# Autodesk Inventor assembly: X Axis Assembly
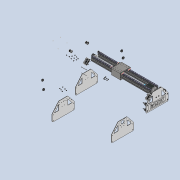
[picture p0: Inventor's stored thumbnail of the model, 180x180]
Saved by Autodesk Inventor 2022 (Build 260153000, 153)
## iProperties
Created: 2021-10-10
Part Number: X Axis Assembly
Document SubType Name: Assembly
Designer: Coy
Author: Coy
## Documents named in this file (23)
- H:\3D Files\Project 3D Models\Breakfast Maker 2000\Assemblys\X Axis Assembly.iam
- H:\3D Files\Project 3D Models\Breakfast Maker 2000\Aluminum Extrusion\2040\2040x700 silver profile.ipt
- H:\3D Files\Project 3D Models\Breakfast Maker 2000\Linear Actuators\MGN12C Linear Rail.iam
- H:\3D Files\Downloaded 3D Files\GrabCad Downloads\hiwin-mgn-series-full-2.snapshot.14\PRODUCT_NAME_10.ipt
- H:\3D Files\Project 3D Models\Breakfast Maker 2000\X Axis V Wheel and Motor Frame Machined.ipt
- H:\3D Files\Project 3D Models\Breakfast Maker 2000\Motors\Nema 23 Dual Shaft 87mm Stepper Motor.ipt
- H:\3D Files\Project 3D Models\Breakfast Maker 2000\X Axis V Wheel Frame Machined.ipt
- H:\3D Files\Project 3D Models\Breakfast Maker 2000\Bearings\0.5in Flanged Pillowblock Frame.ipt
- H:\3D Files\Project 3D Models\Breakfast Maker 2000\Bearings\0.25in ID 0.5in OD 0.1875in Deep Roller Bearing.ipt
- H:\3D Files\Project 3D Models\Breakfast Maker 2000\Shafts and Rods\M6.35 x 356mm Aluminum Rod.ipt
- H:\3D Files\Project 3D Models\Breakfast Maker 2000\Shafts and Rods\M6.35 x 275mm Aluminum Rod.ipt
- H:\3D Files\Project 3D Models\Breakfast Maker 2000\Couplers\M6.35 Rigid Coupler.ipt
- H:\3D Files\Project 3D Models\Breakfast Maker 2000\Pullys\M6.35 24Tooth 15mm Deep 3M Timing Pulley.ipt
- H:\3D Files\Project 3D Models\Breakfast Maker 2000\3in x 5in Steel Rectangular Tubing 4in long.ipt
- H:\3D Files\Project 3D Models\Breakfast Maker 2000\Pullys\8mm ID 15mm Deep Idler Pully.ipt
- H:\3D Files\Project 3D Models\Breakfast Maker 2000\Bearings\5mm ID 8mm OD 2.5mm Deep Roller Bearing (2021_08_15 23_37_01 UTC).ipt
- H:\3D Files\Project 3D Models\Breakfast Maker 2000\X Axis V Wheel Outside Frame Machined.ipt
- H:\3D Files\Project 3D Models\Breakfast Maker 2000\Shafts and Rods\M5 55mm Threaded Rod.ipt
- H:\3D Files\Project 3D Models\Breakfast Maker 2000\X Axis Belt and V Wheel Plate Spacer.ipt
- H:\3D Files\Project 3D Models\Breakfast Maker 2000\Nuts and Bolts\M5 Nut Silver.ipt
- H:\3D Files\Project 3D Models\Breakfast Maker 2000\Idler Pully Spacer.ipt
- H:\3D Files\Project 3D Models\Breakfast Maker 2000\V Wheel Spacer.ipt
- H:\3D Files\Project 3D Models\Breakfast Maker 2000\M5 V Wheel.ipt
## Components (154 placed, 22 different names)
1. 2040x700 silver profile:1 — Flush:1, Flush:2, Mate:2, Mate:4, Flush:6
2. 2040x700 silver profile:2 — Mate:1, Flush:1, Flush:2, Mate:2, Mate:3, Flush:3, Flush:4, Mate:43
3. MGN12C Linear Rail:1 [sub-assembly] — Mate:7, Flush:11, Flush:12, Mate:9, Flush:15, Flush:16, Mate:42
4. MGN12C Linear Rail:2 [sub-assembly] — Mate:8, Flush:13, Flush:14, Mate:10, Flush:17, Flush:18
5. MGN12C Linear Rail:3 [sub-assembly] — Mate:10, Flush:17, Flush:18, Mate:12, Flush:21, Flush:22
6. MGN12C Linear Rail:4 [sub-assembly] — Mate:9, Flush:15, Flush:16, Mate:11, Flush:19, Flush:20
7. PRODUCT_NAME_10:1 — Mate:6, Flush:9, Flush:10, Mate:8, Flush:13, Flush:14
8. PRODUCT_NAME_10:2 — Mate:4, Flush:5, Flush:6, Mate:6, Flush:9, Flush:10
9. PRODUCT_NAME_10:3 — Mate:11, Flush:19, Flush:20, Mate:13, Flush:23, Flush:24
10. PRODUCT_NAME_10:4 — Mate:12, Flush:21, Flush:22, Mate:14, Flush:25, Flush:26
11. PRODUCT_NAME_10:5 — Mate:13, Flush:23, Flush:24, Mate:15, Flush:27, Flush:28
12. PRODUCT_NAME_10:6 — Mate:14, Flush:25, Flush:26, Mate:16, Flush:29, Flush:30
13. PRODUCT_NAME_10:7 — Mate:16, Flush:29, Flush:30
14. PRODUCT_NAME_10:8 — Mate:15, Flush:27, Flush:28
15. PRODUCT_NAME_10:9 — Mate:3, Flush:3, Flush:4, Flush:5, Flush:7, Flush:8, Mate:5
16. PRODUCT_NAME_10:10 — Flush:7, Flush:8, Mate:5, Mate:7, Flush:11, Flush:12
17. Nema 23 Dual Shaft 87mm Stepper Motor:1 — Mate:30, Mate:31, Mate:37, Mate:38, Mate:39, Mate:181
18. 0.5in Flanged Pillowblock Frame:1 — Mate:29, Flush:31
19. 0.25in ID 0.5in OD 0.1875in Deep Roller Bearing:1 — Mate:29, Flush:31
20. M6.35 x 356mm Aluminum Rod:1 — Mate:30, Mate:31, Mate:32, Mate:33, Mate:36
21. M6.35 x 275mm Aluminum Rod:1 — Mate:32, Mate:33, Mate:34, Mate:35, Mate:40
22. M6.35 Rigid Coupler:1 — Mate:34, Mate:35
23. M6.35 Rigid Coupler:2 — Mate:36, Mate:37
24. M6.35 24Tooth 15mm Deep 3M Timing Pulley:1 — Mate:38, Mate:39
25. M6.35 24Tooth 15mm Deep 3M Timing Pulley:2 — Mate:40
26. 3in x 5in Steel Rectangular Tubing 4in long:1 — Mate:42, Mate:43
27. 8mm ID 15mm Deep Idler Pully:1 — Mate:45, Mate:46, Flush:35, Flush:36
28. 8mm ID 15mm Deep Idler Pully:2 — Mate:44, Flush:32, Mate:47, Flush:39
29. 8mm ID 15mm Deep Idler Pully:3 — Mate:48, Mate:51, Flush:33, Flush:37
30. 8mm ID 15mm Deep Idler Pully:4 — Mate:49, Mate:50, Flush:34, Flush:38
31. 5mm ID 8mm OD 2.5mm Deep Roller Bearing (2021_08_15 23_37_01 UTC):1 — Mate:44, Flush:32, Mate:102, Mate:112
32. 5mm ID 8mm OD 2.5mm Deep Roller Bearing (2021_08_15 23_37_01 UTC):2 — Mate:47, Flush:39, Mate:108
33. 5mm ID 8mm OD 2.5mm Deep Roller Bearing (2021_08_15 23_37_01 UTC):3 — Mate:46, Flush:36, Mate:107
34. 5mm ID 8mm OD 2.5mm Deep Roller Bearing (2021_08_15 23_37_01 UTC):4 — Mate:45, Flush:35, Mate:101, Mate:111
35. 5mm ID 8mm OD 2.5mm Deep Roller Bearing (2021_08_15 23_37_01 UTC):5 — Mate:51, Flush:33
36. 5mm ID 8mm OD 2.5mm Deep Roller Bearing (2021_08_15 23_37_01 UTC):6 — Mate:48, Flush:37
37. 5mm ID 8mm OD 2.5mm Deep Roller Bearing (2021_08_15 23_37_01 UTC):7 — Mate:49, Flush:38
38. 5mm ID 8mm OD 2.5mm Deep Roller Bearing (2021_08_15 23_37_01 UTC):8 — Mate:50, Flush:34
39. X Axis V Wheel Outside Frame Machined:1
40. X Axis V Wheel Outside Frame Machined:2 — Mate:165, Mate:166, Mate:167, Mate:178
41. M5 55mm Threaded Rod:1 — Mate:90, Mate:98, Mate:120, Mate:128, Mate:136, Mate:143, Mate:151, Mate:159, Mate:171
42. M5 55mm Threaded Rod:2 — Mate:84, Mate:95, Mate:118, Mate:125, Mate:134, Mate:141, Mate:150, Mate:158, Mate:168
43. M5 55mm Threaded Rod:3 — Mate:91, Mate:99, Mate:119, Mate:127, Mate:135, Mate:144, Mate:152, Mate:160, Mate:165, Mate:169
44. M5 55mm Threaded Rod:4 — Mate:85, Mate:94, Mate:117, Mate:126, Mate:133, Mate:142, Mate:149, Mate:157, Mate:166, Mate:170
45. M5 55mm Threaded Rod:5 — Mate:96, Mate:102, Mate:103, Mate:110, Mate:114, Mate:174, Mate:179
46. M5 55mm Threaded Rod:6 — Mate:97, Mate:101, Mate:104, Mate:109, Mate:113, Mate:175, Mate:180
47. M5 55mm Threaded Rod:7
48. M5 55mm Threaded Rod:8
49. M5 55mm Threaded Rod:9
50. M5 55mm Threaded Rod:10
51. M5 55mm Threaded Rod:11
52. M5 55mm Threaded Rod:12
53. X Axis Belt and V Wheel Plate Spacer:1 — Mate:72, Mate:73, Mate:167
54. X Axis Belt and V Wheel Plate Spacer:2 — Mate:74, Mate:75
55. X Axis Belt and V Wheel Plate Spacer:3 — Mate:76, Mate:77
56. X Axis Belt and V Wheel Plate Spacer:4 — Mate:78, Mate:79
57. M5 55mm Threaded Rod:13 — Mate:72, Mate:87, Mate:172
58. M5 55mm Threaded Rod:14 — Mate:73, Mate:86, Mate:173
59. M5 55mm Threaded Rod:15 — Mate:76
60. M5 55mm Threaded Rod:16 — Mate:79
61. M5 55mm Threaded Rod:17 — Mate:75, Mate:89, Mate:176
62. M5 55mm Threaded Rod:18 — Mate:74, Mate:88, Mate:177
63. M5 55mm Threaded Rod:19 — Mate:77
64. M5 55mm Threaded Rod:20 — Mate:78
65. M5 Nut Silver:1 — Mate:86, Flush:63
66. M5 Nut Silver:2 — Mate:95, Flush:66, Mate:122
67. M5 Nut Silver:3 — Mate:87, Flush:63, Flush:64, Flush:65
68. M5 Nut Silver:4 — Mate:89, Flush:60
69. M5 Nut Silver:5 — Mate:88, Flush:60, Flush:61, Flush:62
70. M5 Nut Silver:6 — Mate:90, Flush:61
71. M5 Nut Silver:7 — Mate:85, Flush:64
72. M5 Nut Silver:8 — Mate:91, Flush:62
73. M5 Nut Silver:9 — Mate:94, Flush:66, Flush:67, Flush:68, Flush:69, Flush:70, Mate:121
74. M5 Nut Silver:10 — Mate:84, Flush:65, Flush:80, Flush:81
75. M5 Nut Silver:11
76. M5 Nut Silver:12
77. M5 Nut Silver:13 — Mate:181
78. M5 Nut Silver:14
79. M5 Nut Silver:15 — Mate:179, Flush:80
80. M5 Nut Silver:16
81. M5 Nut Silver:17
82. M5 Nut Silver:18
83. M5 Nut Silver:19
84. M5 Nut Silver:20 — Mate:180, Flush:81
85. M5 Nut Silver:21 — Mate:96, Flush:67, Mate:105
86. M5 Nut Silver:22 — Mate:97, Flush:68, Mate:106
87. M5 Nut Silver:23 — Mate:98, Flush:69, Mate:123
88. M5 Nut Silver:24 — Mate:171, Flush:78
89. M5 Nut Silver:25 — Mate:170, Flush:71
90. M5 Nut Silver:26 — Mate:99, Flush:70, Mate:124
91. M5 Nut Silver:27 — Mate:177, Flush:76
92. M5 Nut Silver:28 — Mate:175, Flush:75
93. M5 Nut Silver:29 — Mate:172, Flush:73
94. M5 Nut Silver:30 — Mate:176, Flush:77
95. M5 Nut Silver:31 — Mate:174, Flush:74
96. M5 Nut Silver:32 — Mate:173, Flush:72
97. M5 Nut Silver:33 — Mate:141, Mate:146, Mate:156
98. M5 Nut Silver:34 — Mate:142, Mate:145, Mate:155
99. M5 Nut Silver:35 — Mate:143, Mate:147, Mate:154
100. M5 Nut Silver:36 — Mate:157, Mate:161
101. M5 Nut Silver:37 — Mate:158, Mate:162
102. M5 Nut Silver:38 — Mate:144, Mate:148, Mate:153
103. M5 Nut Silver:39 — Mate:159, Mate:163
104. M5 Nut Silver:40 — Mate:168, Mate:178, Flush:71, Flush:72, Flush:73, Flush:74, Flush:75, Flush:76, Flush:77, Flush:78, Flush:79
105. M5 Nut Silver:41 — Mate:160, Mate:164
106. M5 Nut Silver:42 — Mate:169, Flush:79
107. M5 Nut Silver:43
108. M5 Nut Silver:44
109. M5 Nut Silver:45
110. M5 Nut Silver:46
111. M5 Nut Silver:47
112. M5 Nut Silver:48
113. M5 Nut Silver:49
114. M5 Nut Silver:50
115. M5 Nut Silver:51
116. M5 Nut Silver:52
117. M5 Nut Silver:53 — Mate:113, Mate:115
118. M5 Nut Silver:54 — Mate:125, Mate:130, Mate:138
119. M5 Nut Silver:55 — Mate:127, Mate:132, Mate:140
120. M5 Nut Silver:56 — Mate:114, Mate:116
121. M5 Nut Silver:57 — Mate:126, Mate:129, Mate:137
122. M5 Nut Silver:58 — Mate:128, Mate:131, Mate:139
123. M5 Nut Silver:59
124. M5 Nut Silver:60
125. M5 Nut Silver:61
126. M5 Nut Silver:62
127. M5 Nut Silver:63
128. M5 Nut Silver:64
129. Idler Pully Spacer:1 — Mate:104, Mate:106, Mate:107
130. Idler Pully Spacer:2 — Mate:103, Mate:105, Mate:108
131. Idler Pully Spacer:3 — Mate:109, Mate:111, Mate:115
132. Idler Pully Spacer:4 — Mate:110, Mate:112, Mate:116
133. Idler Pully Spacer:5
134. Idler Pully Spacer:6
135. Idler Pully Spacer:7
136. Idler Pully Spacer:8
137. V Wheel Spacer:1 — Mate:117, Mate:121, Mate:129
138. V Wheel Spacer:2 — Mate:118, Mate:122, Mate:130
139. V Wheel Spacer:3 — Mate:149, Mate:155, Mate:161
140. V Wheel Spacer:4 — Mate:150, Mate:156, Mate:162
141. V Wheel Spacer:5 — Mate:120, Mate:123, Mate:131
142. V Wheel Spacer:6 — Mate:151, Mate:154, Mate:163
143. V Wheel Spacer:7 — Mate:119, Mate:124, Mate:132
144. V Wheel Spacer:8 — Mate:152, Mate:153, Mate:164
145. M5 V Wheel:1 — Mate:134, Mate:138, Mate:146
146. M5 V Wheel:2 — Mate:133, Mate:137, Mate:145
147. M5 V Wheel:3 — Mate:135, Mate:140, Mate:148
148. M5 V Wheel:4 — Mate:136, Mate:139, Mate:147
149. M5 V Wheel:5
150. M5 V Wheel:6
151. M5 V Wheel:7
152. M5 V Wheel:8
153. X Axis V Wheel and Motor Frame Machined:1
154. X Axis V Wheel Frame Machined:1
## Relationships (202: Mate 141, Flush 61)
- Mate:1: 2040x700 silver profile:2
- Flush:1: 2040x700 silver profile:1 ↔ 2040x700 silver profile:2
- Flush:2: 2040x700 silver profile:1 ↔ 2040x700 silver profile:2
- Mate:2 (60 mm): 2040x700 silver profile:1 ↔ 2040x700 silver profile:2
- Mate:3: 2040x700 silver profile:2 ↔ PRODUCT_NAME_10:9
- Flush:3 (4 mm): 2040x700 silver profile:2 ↔ PRODUCT_NAME_10:9
- Flush:4: 2040x700 silver profile:2 ↔ PRODUCT_NAME_10:9
- Mate:4: 2040x700 silver profile:1 ↔ PRODUCT_NAME_10:2
- Flush:5: PRODUCT_NAME_10:2 ↔ PRODUCT_NAME_10:9
- Flush:6 (4 mm): 2040x700 silver profile:1 ↔ PRODUCT_NAME_10:2
- Flush:7: PRODUCT_NAME_10:9 ↔ PRODUCT_NAME_10:10
- Flush:8: PRODUCT_NAME_10:9 ↔ PRODUCT_NAME_10:10
- Mate:5: PRODUCT_NAME_10:9 ↔ PRODUCT_NAME_10:10
- Mate:6: PRODUCT_NAME_10:1 ↔ PRODUCT_NAME_10:2
- Flush:9: PRODUCT_NAME_10:1 ↔ PRODUCT_NAME_10:2
- Flush:10: PRODUCT_NAME_10:1 ↔ PRODUCT_NAME_10:2
- Mate:7: MGN12C Linear Rail:1 ↔ PRODUCT_NAME_10:10
- Flush:11: MGN12C Linear Rail:1 ↔ PRODUCT_NAME_10:10
- Flush:12: MGN12C Linear Rail:1 ↔ PRODUCT_NAME_10:10
- Mate:8: MGN12C Linear Rail:2 ↔ PRODUCT_NAME_10:1
- Flush:13: MGN12C Linear Rail:2 ↔ PRODUCT_NAME_10:1
- Flush:14: MGN12C Linear Rail:2 ↔ PRODUCT_NAME_10:1
- Mate:9: MGN12C Linear Rail:1 ↔ MGN12C Linear Rail:4
- Flush:15: MGN12C Linear Rail:1 ↔ MGN12C Linear Rail:4
- Flush:16: MGN12C Linear Rail:1 ↔ MGN12C Linear Rail:4
- Mate:10: MGN12C Linear Rail:2 ↔ MGN12C Linear Rail:3
- Flush:17: MGN12C Linear Rail:2 ↔ MGN12C Linear Rail:3
- Flush:18: MGN12C Linear Rail:2 ↔ MGN12C Linear Rail:3
- Mate:11: MGN12C Linear Rail:4 ↔ PRODUCT_NAME_10:3
- Flush:19: MGN12C Linear Rail:4 ↔ PRODUCT_NAME_10:3
- Flush:20: MGN12C Linear Rail:4 ↔ PRODUCT_NAME_10:3
- Mate:12: MGN12C Linear Rail:3 ↔ PRODUCT_NAME_10:4
- Flush:21: MGN12C Linear Rail:3 ↔ PRODUCT_NAME_10:4
- Flush:22: MGN12C Linear Rail:3 ↔ PRODUCT_NAME_10:4
- Mate:13: PRODUCT_NAME_10:3 ↔ PRODUCT_NAME_10:5
- Flush:23: PRODUCT_NAME_10:3 ↔ PRODUCT_NAME_10:5
- Flush:24: PRODUCT_NAME_10:3 ↔ PRODUCT_NAME_10:5
- Mate:14: PRODUCT_NAME_10:4 ↔ PRODUCT_NAME_10:6
- Flush:25: PRODUCT_NAME_10:4 ↔ PRODUCT_NAME_10:6
- Flush:26: PRODUCT_NAME_10:4 ↔ PRODUCT_NAME_10:6
- Mate:15: PRODUCT_NAME_10:5 ↔ PRODUCT_NAME_10:8
- Flush:27: PRODUCT_NAME_10:5 ↔ PRODUCT_NAME_10:8
- Flush:28: PRODUCT_NAME_10:5 ↔ PRODUCT_NAME_10:8
- Mate:16: PRODUCT_NAME_10:6 ↔ PRODUCT_NAME_10:7
- Flush:29: PRODUCT_NAME_10:6 ↔ PRODUCT_NAME_10:7
- Flush:30: PRODUCT_NAME_10:6 ↔ PRODUCT_NAME_10:7
- Mate:29: 0.5in Flanged Pillowblock Frame:1 ↔ 0.25in ID 0.5in OD 0.1875in Deep Roller Bearing:1
- Flush:31: 0.5in Flanged Pillowblock Frame:1 ↔ 0.25in ID 0.5in OD 0.1875in Deep Roller Bearing:1
- Mate:30: Nema 23 Dual Shaft 87mm Stepper Motor:1 ↔ M6.35 x 356mm Aluminum Rod:1
- Mate:31: Nema 23 Dual Shaft 87mm Stepper Motor:1 ↔ M6.35 x 356mm Aluminum Rod:1
- Mate:32: M6.35 x 356mm Aluminum Rod:1 ↔ M6.35 x 275mm Aluminum Rod:1
- Mate:33: M6.35 x 356mm Aluminum Rod:1 ↔ M6.35 x 275mm Aluminum Rod:1
- Mate:34: M6.35 x 275mm Aluminum Rod:1 ↔ M6.35 Rigid Coupler:1
- Mate:35 (-12.5 mm): M6.35 x 275mm Aluminum Rod:1 ↔ M6.35 Rigid Coupler:1
- Mate:36: M6.35 x 356mm Aluminum Rod:1 ↔ M6.35 Rigid Coupler:2
- Mate:37 (2.5 mm): Nema 23 Dual Shaft 87mm Stepper Motor:1 ↔ M6.35 Rigid Coupler:2
- Mate:38: Nema 23 Dual Shaft 87mm Stepper Motor:1 ↔ M6.35 24Tooth 15mm Deep 3M Timing Pulley:1
- Mate:39 (0.2 mm): Nema 23 Dual Shaft 87mm Stepper Motor:1 ↔ M6.35 24Tooth 15mm Deep 3M Timing Pulley:1
- Mate:40: M6.35 x 275mm Aluminum Rod:1 ↔ M6.35 24Tooth 15mm Deep 3M Timing Pulley:2
- Mate:42: MGN12C Linear Rail:1 ↔ 3in x 5in Steel Rectangular Tubing 4in long:1
- Mate:43 (7.15 mm): 2040x700 silver profile:2 ↔ 3in x 5in Steel Rectangular Tubing 4in long:1
- Mate:44: 8mm ID 15mm Deep Idler Pully:2 ↔ 5mm ID 8mm OD 2.5mm Deep Roller Bearing (2021_08_15 23_37_01 UTC):1
- Flush:32: 8mm ID 15mm Deep Idler Pully:2 ↔ 5mm ID 8mm OD 2.5mm Deep Roller Bearing (2021_08_15 23_37_01 UTC):1
- Mate:45: 8mm ID 15mm Deep Idler Pully:1 ↔ 5mm ID 8mm OD 2.5mm Deep Roller Bearing (2021_08_15 23_37_01 UTC):4
- Mate:46: 8mm ID 15mm Deep Idler Pully:1 ↔ 5mm ID 8mm OD 2.5mm Deep Roller Bearing (2021_08_15 23_37_01 UTC):3
- Mate:47: 8mm ID 15mm Deep Idler Pully:2 ↔ 5mm ID 8mm OD 2.5mm Deep Roller Bearing (2021_08_15 23_37_01 UTC):2
- Mate:48: 8mm ID 15mm Deep Idler Pully:3 ↔ 5mm ID 8mm OD 2.5mm Deep Roller Bearing (2021_08_15 23_37_01 UTC):6
- Mate:49: 8mm ID 15mm Deep Idler Pully:4 ↔ 5mm ID 8mm OD 2.5mm Deep Roller Bearing (2021_08_15 23_37_01 UTC):7
- Mate:50: 8mm ID 15mm Deep Idler Pully:4 ↔ 5mm ID 8mm OD 2.5mm Deep Roller Bearing (2021_08_15 23_37_01 UTC):8
- Mate:51: 8mm ID 15mm Deep Idler Pully:3 ↔ 5mm ID 8mm OD 2.5mm Deep Roller Bearing (2021_08_15 23_37_01 UTC):5
- Flush:33: 8mm ID 15mm Deep Idler Pully:3 ↔ 5mm ID 8mm OD 2.5mm Deep Roller Bearing (2021_08_15 23_37_01 UTC):5
- Flush:34: 8mm ID 15mm Deep Idler Pully:4 ↔ 5mm ID 8mm OD 2.5mm Deep Roller Bearing (2021_08_15 23_37_01 UTC):8
- Flush:35: 8mm ID 15mm Deep Idler Pully:1 ↔ 5mm ID 8mm OD 2.5mm Deep Roller Bearing (2021_08_15 23_37_01 UTC):4
- Flush:36: 8mm ID 15mm Deep Idler Pully:1 ↔ 5mm ID 8mm OD 2.5mm Deep Roller Bearing (2021_08_15 23_37_01 UTC):3
- Flush:37: 8mm ID 15mm Deep Idler Pully:3 ↔ 5mm ID 8mm OD 2.5mm Deep Roller Bearing (2021_08_15 23_37_01 UTC):6
- Flush:38: 8mm ID 15mm Deep Idler Pully:4 ↔ 5mm ID 8mm OD 2.5mm Deep Roller Bearing (2021_08_15 23_37_01 UTC):7
- Flush:39: 8mm ID 15mm Deep Idler Pully:2 ↔ 5mm ID 8mm OD 2.5mm Deep Roller Bearing (2021_08_15 23_37_01 UTC):2
- Mate:72: X Axis Belt and V Wheel Plate Spacer:1 ↔ M5 55mm Threaded Rod:13
- Mate:73: X Axis Belt and V Wheel Plate Spacer:1 ↔ M5 55mm Threaded Rod:14
- Mate:74: X Axis Belt and V Wheel Plate Spacer:2 ↔ M5 55mm Threaded Rod:18
- Mate:75: X Axis Belt and V Wheel Plate Spacer:2 ↔ M5 55mm Threaded Rod:17
- Mate:76: X Axis Belt and V Wheel Plate Spacer:3 ↔ M5 55mm Threaded Rod:15
- Mate:77: X Axis Belt and V Wheel Plate Spacer:3 ↔ M5 55mm Threaded Rod:19
- Mate:78: X Axis Belt and V Wheel Plate Spacer:4 ↔ M5 55mm Threaded Rod:20
- Mate:79: X Axis Belt and V Wheel Plate Spacer:4 ↔ M5 55mm Threaded Rod:16
- Mate:84: M5 55mm Threaded Rod:2 ↔ M5 Nut Silver:10
- Mate:85: M5 55mm Threaded Rod:4 ↔ M5 Nut Silver:7
- Mate:86: M5 55mm Threaded Rod:14 ↔ M5 Nut Silver:1
- Mate:87: M5 55mm Threaded Rod:13 ↔ M5 Nut Silver:3
- Mate:88: M5 55mm Threaded Rod:18 ↔ M5 Nut Silver:5
- Mate:89: M5 55mm Threaded Rod:17 ↔ M5 Nut Silver:4
- Mate:90: M5 55mm Threaded Rod:1 ↔ M5 Nut Silver:6
- Mate:91: M5 55mm Threaded Rod:3 ↔ M5 Nut Silver:8
- Flush:60: M5 Nut Silver:4 ↔ M5 Nut Silver:5
- Flush:61: M5 Nut Silver:5 ↔ M5 Nut Silver:6
- Flush:62: M5 Nut Silver:5 ↔ M5 Nut Silver:8
- Flush:63: M5 Nut Silver:1 ↔ M5 Nut Silver:3
- Flush:64: M5 Nut Silver:3 ↔ M5 Nut Silver:7
- Flush:65: M5 Nut Silver:3 ↔ M5 Nut Silver:10
- Mate:94: M5 55mm Threaded Rod:4 ↔ M5 Nut Silver:9
- Mate:95: M5 55mm Threaded Rod:2 ↔ M5 Nut Silver:2
- Mate:96: M5 55mm Threaded Rod:5 ↔ M5 Nut Silver:21
- Mate:97: M5 55mm Threaded Rod:6 ↔ M5 Nut Silver:22
- Mate:98: M5 55mm Threaded Rod:1 ↔ M5 Nut Silver:23
- Mate:99: M5 55mm Threaded Rod:3 ↔ M5 Nut Silver:26
- Flush:66: M5 Nut Silver:2 ↔ M5 Nut Silver:9
- Flush:67: M5 Nut Silver:9 ↔ M5 Nut Silver:21
- Flush:68: M5 Nut Silver:9 ↔ M5 Nut Silver:22
- Flush:69: M5 Nut Silver:9 ↔ M5 Nut Silver:23
- Flush:70: M5 Nut Silver:9 ↔ M5 Nut Silver:26
- Mate:101: 5mm ID 8mm OD 2.5mm Deep Roller Bearing (2021_08_15 23_37_01 UTC):4 ↔ M5 55mm Threaded Rod:6
- Mate:102: 5mm ID 8mm OD 2.5mm Deep Roller Bearing (2021_08_15 23_37_01 UTC):1 ↔ M5 55mm Threaded Rod:5
- Mate:103: M5 55mm Threaded Rod:5 ↔ Idler Pully Spacer:2
- Mate:104: M5 55mm Threaded Rod:6 ↔ Idler Pully Spacer:1
- Mate:105: M5 Nut Silver:21 ↔ Idler Pully Spacer:2
- Mate:106: M5 Nut Silver:22 ↔ Idler Pully Spacer:1
- Mate:107: 5mm ID 8mm OD 2.5mm Deep Roller Bearing (2021_08_15 23_37_01 UTC):3 ↔ Idler Pully Spacer:1
- Mate:108: 5mm ID 8mm OD 2.5mm Deep Roller Bearing (2021_08_15 23_37_01 UTC):2 ↔ Idler Pully Spacer:2
- Mate:109: M5 55mm Threaded Rod:6 ↔ Idler Pully Spacer:3
- Mate:110: M5 55mm Threaded Rod:5 ↔ Idler Pully Spacer:4
- Mate:111: 5mm ID 8mm OD 2.5mm Deep Roller Bearing (2021_08_15 23_37_01 UTC):4 ↔ Idler Pully Spacer:3
- Mate:112: 5mm ID 8mm OD 2.5mm Deep Roller Bearing (2021_08_15 23_37_01 UTC):1 ↔ Idler Pully Spacer:4
- Mate:113: M5 55mm Threaded Rod:6 ↔ M5 Nut Silver:53
- Mate:114: M5 55mm Threaded Rod:5 ↔ M5 Nut Silver:56
- Mate:115: M5 Nut Silver:53 ↔ Idler Pully Spacer:3
- Mate:116: M5 Nut Silver:56 ↔ Idler Pully Spacer:4
- Mate:117: M5 55mm Threaded Rod:4 ↔ V Wheel Spacer:1
- Mate:118: M5 55mm Threaded Rod:2 ↔ V Wheel Spacer:2
- Mate:119: M5 55mm Threaded Rod:3 ↔ V Wheel Spacer:7
- Mate:120: M5 55mm Threaded Rod:1 ↔ V Wheel Spacer:5
- Mate:121: M5 Nut Silver:9 ↔ V Wheel Spacer:1
- Mate:122: M5 Nut Silver:2 ↔ V Wheel Spacer:2
- Mate:123: M5 Nut Silver:23 ↔ V Wheel Spacer:5
- Mate:124: M5 Nut Silver:26 ↔ V Wheel Spacer:7
- Mate:125: M5 55mm Threaded Rod:2 ↔ M5 Nut Silver:54
- Mate:126: M5 55mm Threaded Rod:4 ↔ M5 Nut Silver:57
- Mate:127: M5 55mm Threaded Rod:3 ↔ M5 Nut Silver:55
- Mate:128: M5 55mm Threaded Rod:1 ↔ M5 Nut Silver:58
- Mate:129: M5 Nut Silver:57 ↔ V Wheel Spacer:1
- Mate:130: M5 Nut Silver:54 ↔ V Wheel Spacer:2
- Mate:131: M5 Nut Silver:58 ↔ V Wheel Spacer:5
- Mate:132: M5 Nut Silver:55 ↔ V Wheel Spacer:7
- Mate:133: M5 55mm Threaded Rod:4 ↔ M5 V Wheel:2
- Mate:134: M5 55mm Threaded Rod:2 ↔ M5 V Wheel:1
- Mate:135: M5 55mm Threaded Rod:3 ↔ M5 V Wheel:3
- Mate:136: M5 55mm Threaded Rod:1 ↔ M5 V Wheel:4
- Mate:137: M5 Nut Silver:57 ↔ M5 V Wheel:2
- Mate:138: M5 Nut Silver:54 ↔ M5 V Wheel:1
- Mate:139: M5 Nut Silver:58 ↔ M5 V Wheel:4
- Mate:140: M5 Nut Silver:55 ↔ M5 V Wheel:3
- Mate:141: M5 55mm Threaded Rod:2 ↔ M5 Nut Silver:33
- Mate:142: M5 55mm Threaded Rod:4 ↔ M5 Nut Silver:34
- Mate:143: M5 55mm Threaded Rod:1 ↔ M5 Nut Silver:35
- Mate:144: M5 55mm Threaded Rod:3 ↔ M5 Nut Silver:38
- Mate:145: M5 Nut Silver:34 ↔ M5 V Wheel:2
- Mate:146: M5 Nut Silver:33 ↔ M5 V Wheel:1
- Mate:147: M5 Nut Silver:35 ↔ M5 V Wheel:4
- Mate:148: M5 Nut Silver:38 ↔ M5 V Wheel:3
- Mate:149: M5 55mm Threaded Rod:4 ↔ V Wheel Spacer:3
- Mate:150: M5 55mm Threaded Rod:2 ↔ V Wheel Spacer:4
- Mate:151: M5 55mm Threaded Rod:1 ↔ V Wheel Spacer:6
- Mate:152: M5 55mm Threaded Rod:3 ↔ V Wheel Spacer:8
- Mate:153: M5 Nut Silver:38 ↔ V Wheel Spacer:8
- Mate:154: M5 Nut Silver:35 ↔ V Wheel Spacer:6
- Mate:155: M5 Nut Silver:34 ↔ V Wheel Spacer:3
- Mate:156: M5 Nut Silver:33 ↔ V Wheel Spacer:4
- Mate:157: M5 55mm Threaded Rod:4 ↔ M5 Nut Silver:36
- Mate:158: M5 55mm Threaded Rod:2 ↔ M5 Nut Silver:37
- Mate:159: M5 55mm Threaded Rod:1 ↔ M5 Nut Silver:39
- Mate:160: M5 55mm Threaded Rod:3 ↔ M5 Nut Silver:41
- Mate:161: M5 Nut Silver:36 ↔ V Wheel Spacer:3
- Mate:162: M5 Nut Silver:37 ↔ V Wheel Spacer:4
- Mate:163: M5 Nut Silver:39 ↔ V Wheel Spacer:6
- Mate:164: M5 Nut Silver:41 ↔ V Wheel Spacer:8
- Mate:165: X Axis V Wheel Outside Frame Machined:2 ↔ M5 55mm Threaded Rod:3
- Mate:166: X Axis V Wheel Outside Frame Machined:2 ↔ M5 55mm Threaded Rod:4
- Mate:167 (0.025 mm): X Axis V Wheel Outside Frame Machined:2 ↔ X Axis Belt and V Wheel Plate Spacer:1
- Mate:168: M5 55mm Threaded Rod:2 ↔ M5 Nut Silver:40
- Mate:169: M5 55mm Threaded Rod:3 ↔ M5 Nut Silver:42
- Mate:170: M5 55mm Threaded Rod:4 ↔ M5 Nut Silver:25
- Mate:171: M5 55mm Threaded Rod:1 ↔ M5 Nut Silver:24
- Mate:172: M5 55mm Threaded Rod:13 ↔ M5 Nut Silver:29
- Mate:173: M5 55mm Threaded Rod:14 ↔ M5 Nut Silver:32
- Mate:174: M5 55mm Threaded Rod:5 ↔ M5 Nut Silver:31
- Mate:175: M5 55mm Threaded Rod:6 ↔ M5 Nut Silver:28
- Mate:176: M5 55mm Threaded Rod:17 ↔ M5 Nut Silver:30
- Mate:177: M5 55mm Threaded Rod:18 ↔ M5 Nut Silver:27
- Mate:178: X Axis V Wheel Outside Frame Machined:2 ↔ M5 Nut Silver:40
- Flush:71: M5 Nut Silver:25 ↔ M5 Nut Silver:40
- Flush:72: M5 Nut Silver:32 ↔ M5 Nut Silver:40
- Flush:73: M5 Nut Silver:29 ↔ M5 Nut Silver:40
- Flush:74: M5 Nut Silver:31 ↔ M5 Nut Silver:40
- Flush:75: M5 Nut Silver:28 ↔ M5 Nut Silver:40
- Flush:76: M5 Nut Silver:27 ↔ M5 Nut Silver:40
- Flush:77: M5 Nut Silver:30 ↔ M5 Nut Silver:40
- Flush:78: M5 Nut Silver:24 ↔ M5 Nut Silver:40
- Flush:79: M5 Nut Silver:40 ↔ M5 Nut Silver:42
- Mate:179: M5 55mm Threaded Rod:5 ↔ M5 Nut Silver:15
- Mate:180: M5 55mm Threaded Rod:6 ↔ M5 Nut Silver:20
- Flush:80: M5 Nut Silver:10 ↔ M5 Nut Silver:15
- Flush:81: M5 Nut Silver:10 ↔ M5 Nut Silver:20
- Mate:181: Nema 23 Dual Shaft 87mm Stepper Motor:1 ↔ M5 Nut Silver:13
